# Autodesk Inventor assembly: 90-Degree-Metal-Brace
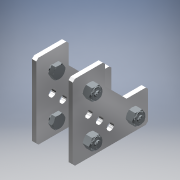
[picture p0: Inventor's stored thumbnail of the model, 180x180]
Saved by Autodesk Inventor 2017.3 (Build 213256000, 256)
## iProperties
Created: 2018-01-05
Part Number: 90-Degree-Metal-Brace
Document SubType Name: Assembly
Designer: pranav
Author: pranav
## iProperties of the stored document REV-41-1361 Simple.ipt
Created: 2017-04-10
Part Number: REV-41-1361 Simple
Material: Generic
Document SubType Name: Modeling
Designer: pranav
Density: 1 g/cm^3
Appearance: Default
Sending System: Autodesk Translation Framework v5.2.0.2920
Preprocessor: ST-DEVELOPER v16.5
Title: E:/Dropbox/REV Robotics/STEP Files/REV-41-1361 Simple.step
## iProperties of the stored document REV-41-1019.ipt
Created: 2015-08-20
Part Number: REV-41-1019
Material: Generic
Description: STEP AP214
Document SubType Name: Modeling
Designer: pranav
Density: 1 g/cm^3
Appearance: Default
Sending System: SolidWorks 2014
Preprocessor: SwSTEP 2.0
Title: REV-41-1019_10mm.STEP
Revision Number: ANY
## iProperties of the stored document REV-41-1359 Simple.ipt
Created: 2017-04-10
Part Number: REV-41-1359 Simple
Material: Generic
Document SubType Name: Modeling
Designer: pranav
Density: 1 g/cm^3
Appearance: Default
Sending System: Autodesk Translation Framework v5.2.0.2920
Preprocessor: ST-DEVELOPER v16.5
Title: E:/Dropbox/REV Robotics/STEP Files/REV-41-1359 Simple.step
## Documents named in this file (7)
- **C:\Users\pranav\Documents\Inventor\REV-Robot-CAD\90-Degree-Metal-Brace.iam*LocalDocs*xPrzvq4shWed3emkkWbjtxzrqNd*REV-41-1361 Simple.ipt
- **C:\Users\pranav\Documents\Inventor\REV-Robot-CAD\90-Degree-Metal-Brace.iam*LocalDocs*xIspevg2yVka0uvkjD3yepuru4c*REV-41-1019.ipt
- **C:\Users\pranav\Documents\Inventor\REV-Robot-CAD\90-Degree-Metal-Brace.iam*LocalDocs*xS5alrn1gO5ure0w5Err235yoGf*REV-41-1359 Simple.ipt
- C:\Users\pranav\Documents\Inventor\REV-Robot-CAD\90-Degree-Metal-Brace.iam
- C:\Users\pranav\Documents\Inventor\REV-Robot-CAD\REV Robotics\REV Robotics CAD\REV-41-1019.STEP
- C:\Users\pranav\Documents\Inventor\REV-Robot-CAD\REV Robotics\REV Robotics CAD\REV-41-1361 Simple.step
- C:\Users\pranav\Documents\Inventor\REV-Robot-CAD\REV Robotics\REV Robotics CAD\REV-41-1359 Simple.step
## Components (14 placed, 3 different names)
1. REV-41-1019:1 — Mate:13, Mate:14, Mate:15, Mate:16, Mate:17, Mate:18
2. REV-41-1019:2 — Mate:8, Mate:9, Mate:11, Mate:19, Mate:20, Mate:21
3. REV-41-1361 Simple:1 — Mate:21, Mate:24
4. REV-41-1361 Simple:2 — Mate:19, Mate:22
5. REV-41-1361 Simple:3 — Mate:16, Mate:25
6. REV-41-1361 Simple:4 — Mate:18, Mate:26
7. REV-41-1361 Simple:5 — Mate:17, Mate:27
8. REV-41-1361 Simple:6 — Mate:20, Mate:23
9. REV-41-1359 Simple:1 — Mate:9, Mate:24
10. REV-41-1359 Simple:2 — Mate:13, Mate:26
11. REV-41-1359 Simple:3 — Mate:14, Mate:25
12. REV-41-1359 Simple:4 — Mate:8, Mate:23
13. REV-41-1359 Simple:5 — Mate:15, Mate:27
14. REV-41-1359 Simple:6 — Mate:11, Mate:22
## Relationships (18: Mate 18)
- Mate:8: REV-41-1019:2 ↔ REV-41-1359 Simple:4
- Mate:9: REV-41-1019:2 ↔ REV-41-1359 Simple:1
- Mate:11: REV-41-1019:2 ↔ REV-41-1359 Simple:6
- Mate:13: REV-41-1019:1 ↔ REV-41-1359 Simple:2
- Mate:14: REV-41-1019:1 ↔ REV-41-1359 Simple:3
- Mate:15: REV-41-1019:1 ↔ REV-41-1359 Simple:5
- Mate:16: REV-41-1019:1 ↔ REV-41-1361 Simple:3
- Mate:17: REV-41-1019:1 ↔ REV-41-1361 Simple:5
- Mate:18: REV-41-1019:1 ↔ REV-41-1361 Simple:4
- Mate:19: REV-41-1019:2 ↔ REV-41-1361 Simple:2
- Mate:20: REV-41-1019:2 ↔ REV-41-1361 Simple:6
- Mate:21: REV-41-1019:2 ↔ REV-41-1361 Simple:1
- Mate:22: REV-41-1361 Simple:2 ↔ REV-41-1359 Simple:6
- Mate:23: REV-41-1361 Simple:6 ↔ REV-41-1359 Simple:4
- Mate:24: REV-41-1361 Simple:1 ↔ REV-41-1359 Simple:1
- Mate:25: REV-41-1361 Simple:3 ↔ REV-41-1359 Simple:3
- Mate:26: REV-41-1361 Simple:4 ↔ REV-41-1359 Simple:2
- Mate:27: REV-41-1361 Simple:5 ↔ REV-41-1359 Simple:5
